# Autodesk Inventor assembly: Assembly
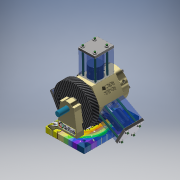
[picture p0: Inventor's stored thumbnail of the model, 180x180]
Saved by Autodesk Inventor 2017 (Build 210142000, 142)
## iProperties
Created: 2020-01-14
Part Number: Assembly
Document SubType Name: Assembly
Designer: Admin
Author: Admin
## Documents named in this file (26)
- D:\tech design 11\Radial Engine\Submission\Parts and Assembly\Assembly23.iam
- D:\tech design 11\Radial Engine\Submission\Parts and Assembly\crankcase.ipt
- D:\tech design 11\Radial Engine\Submission\Parts and Assembly\valve.ipt
- D:\tech design 11\Radial Engine\Submission\Parts and Assembly\valvecrank.ipt
- D:\tech design 11\Radial Engine\Submission\Parts and Assembly\valvehousing.ipt
- D:\tech design 11\Radial Engine\Submission\Parts and Assembly\locatingpin.ipt
- D:\tech design 11\Radial Engine\Submission\Parts and Assembly\cylinder...ipt
- D:\tech design 11\Radial Engine\Submission\Parts and Assembly\base.ipt
- D:\tech design 11\Radial Engine\Submission\Parts and Assembly\bearing.ipt
- D:\tech design 11\Radial Engine\Submission\Parts and Assembly\crankshaft.ipt
- D:\tech design 11\Radial Engine\Submission\Parts and Assembly\flywheel.ipt
- D:\tech design 11\Radial Engine\Assembly\hubpin.ipt
- D:\tech design 11\Radial Engine\Submission\Parts and Assembly\Piston.ipt
- D:\tech design 11\Radial Engine\Submission\Parts and Assembly\Crankcase Cover.ipt
- D:\tech design 11\Radial Engine\Submission\Parts and Assembly\Connecting Rod Hub.ipt
- D:\tech design 11\Radial Engine\Submission\Parts and Assembly\Connecting Rod.ipt
- D:\tech design 11\Radial Engine\Submission\Parts and Assembly\Wrist Pin.ipt
- D:\tech design 11\Radial Engine\Submission\Parts and Assembly\cylinderhead.ipt
- D:\tech design 11\Radial Engine\Submission\Parts and Assembly\enginefoot.ipt
- D:\tech design 11\Radial Engine\Submission\Parts and Assembly\studs.ipt
- D:\tech design 11\Radial Engine\parts\turningfixture.ipt
- D:\tech design 11\Radial Engine\Submission\Parts and Assembly\ventplug.ipt
- C:\Users\Admin\Documents\Inventor\Content Center Files\R2017\en-US\GB_T 70.1-2000\Screw GB_T 70.1 M3 x 14.ipt
- C:\Users\Admin\Documents\Inventor\Content Center Files\R2017\en-US\GB_T 70.1-2000\Screw GB_T 70.1 M3 x 5.ipt
- C:\Users\Admin\Documents\Inventor\Content Center Files\R2017\en-US\PN-87 M-82302\PN-87_M-82302 - M2 x 12.ipt
- C:\Users\Admin\Documents\Inventor\Content Center Files\R2017\en-US\CNS 3129\CNS 3129 - M 2 x 0.4.ipt
## Components (72 placed, 25 different names)
1. crankcase:1 — Insert:2, Insert:3, Insert:4, Insert:5, Insert:6, Insert:7, Mate:4, Insert:27, Mate:17, Insert:33, Insert:34, Mate:18, Mate:19, Insert:50, Mate:44
2. cylinder..:1 — Insert:2, Insert:3, Mate:11, Insert:19, Mate:14
3. cylinder..:2 — Insert:4, Insert:5, Mate:7, Insert:21, Mate:16
4. cylinder..:3 — Insert:6, Insert:7, Mate:5, Insert:20, Mate:15
5. base:1 — Mate:1, Insert:11, Insert:12, Mate:20, Mate:21, Mate:22, Mate:23, Mate:24, Mate:25, Mate:26, Mate:27
6. bearing:1 — Mate:1, Insert:11, Insert:12, Mate:2
7. crankshaft:1 — Mate:2, Mate:4, Rotation:1, Mate:42, Insert:72, Insert:73
8. Crankcase Cover:1 — Mate:19, Insert:51, Insert:52, Insert:53, Insert:54, Insert:55, Insert:56, Mate:44, Insert:72, Insert:74
9. Connecting Rod Hub:1 — Insert:68, Insert:69, Mate:42, Mate:43, Insert:70, Insert:71, Insert:73, Insert:75, Insert:76
10. Connecting Rod:1 — Cylindrical:3, Insert:69
11. Connecting Rod:2 — Cylindrical:1, Insert:68
12. Connecting Rod:3 — Cylindrical:2, Insert:70
13. Piston:1 — Mate:5, Mate:6, Mate:10
14. Piston:2 — Mate:7, Mate:8, Mate:9
15. Piston:3 — Mate:11, Mate:12, Mate:13
16. Wrist Pin:1 — Cylindrical:2, Mate:8, Mate:9
17. Wrist Pin:2 — Cylindrical:1, Mate:6, Mate:10
18. Wrist Pin:3 — Cylindrical:3, Mate:12, Mate:13
19. cylinderhead:1 — Insert:19, Mate:14, Insert:35, Insert:36, Insert:37, Insert:38, Insert:64, Insert:65, Insert:66, Insert:67
20. cylinderhead:2 — Insert:20, Mate:15, Insert:39, Insert:40, Insert:41, Insert:42, Mate:41, Insert:57, Insert:58, Insert:59
21. cylinderhead:3 — Insert:21, Mate:16, Insert:43, Insert:44, Insert:45, Insert:46, Insert:60, Insert:61, Insert:62, Insert:63
22. flywheel:1 — Rotation:1, Insert:74
23. valvecrank:1 — Insert:31, Mate:18, Insert:71
24. hubpin:1 — Mate:43
25. hubpin:2
26. hubpin:3 — Insert:75
27. enginefoot:1 — Insert:50
28. locatingpin:1 — Insert:47
29. studs:1 — Insert:37
30. valve:2 — Insert:31
31. valvehousing:1 — Mate:17, Insert:33, Insert:34, Insert:47, Mate:28, Mate:29, Mate:30, Mate:31, Mate:32, Mate:33, Mate:34, Mate:35, Mate:36, Mate:37, Mate:38, Mate:39
32. ventplug:1 — Insert:27
33. studs:2 — Insert:36
34. studs:3 — Insert:35
35. studs:4 — Insert:39, Mate:40
36. studs:5 — Insert:41
37. studs:6 — Insert:42
38. studs:10 — Insert:38
39. studs:11 — Insert:40
40. studs:12 — Insert:43
41. studs:13 — Insert:45
42. studs:17 — Insert:46
43. studs:19 — Insert:44
44. turningfixture:1
45. Screw GB/T 70.1-2000 M3 x 14:1 — Mate:20, Mate:21
46. Screw GB/T 70.1-2000 M3 x 14:2 — Mate:22, Mate:23
47. Screw GB/T 70.1-2000 M3 x 14:3 — Mate:24, Mate:25
48. Screw GB/T 70.1-2000 M3 x 5:1 — Mate:26, Mate:27
49. PN-87/M-82302 M2 x 12:1 — Mate:28, Mate:29
50. PN-87/M-82302 M2 x 12:2 — Mate:30, Mate:31
51. PN-87/M-82302 M2 x 12:3 — Mate:32, Mate:33
52. PN-87/M-82302 M2 x 12:4 — Mate:34, Mate:35
53. PN-87/M-82302 M2 x 12:5 — Mate:36, Mate:37
54. PN-87/M-82302 M2 x 12:6 — Mate:38, Mate:39
55. PN-87/M-82302 M2 x 12:7 — Insert:51
56. PN-87/M-82302 M2 x 12:8 — Insert:54
57. PN-87/M-82302 M2 x 12:9 — Insert:52
58. PN-87/M-82302 M2 x 12:11 — Insert:56
59. PN-87/M-82302 M2 x 12:12 — Insert:55, Insert:76
60. PN-87/M-82302 M2 x 12:13 — Insert:53
61. CNS 3129 M 2:1 — Mate:40, Mate:41
62. CNS 3129 M 2:2 — Insert:57
63. CNS 3129 M 2:3 — Insert:58
64. CNS 3129 M 2:4 — Insert:59
65. CNS 3129 M 2:5 — Insert:60
66. CNS 3129 M 2:6 — Insert:61
67. CNS 3129 M 2:7 — Insert:62
68. CNS 3129 M 2:8 — Insert:63
69. CNS 3129 M 2:9 — Insert:64
70. CNS 3129 M 2:10 — Insert:65
71. CNS 3129 M 2:11 — Insert:66
72. CNS 3129 M 2:12 — Insert:67
## Relationships (102: Insert 55, Mate 43, CylindricalJoint 3, RelateRotation 1)
- Insert:2: crankcase:1 ↔ cylinder..:1
- Insert:3: crankcase:1 ↔ cylinder..:1
- Insert:4: crankcase:1 ↔ cylinder..:2
- Insert:5: crankcase:1 ↔ cylinder..:2
- Insert:6: crankcase:1 ↔ cylinder..:3
- Insert:7: crankcase:1 ↔ cylinder..:3
- Mate:1: base:1 ↔ bearing:1
- Insert:11: base:1 ↔ bearing:1
- Insert:12: base:1 ↔ bearing:1
- Mate:2: bearing:1 ↔ crankshaft:1
- Mate:4: crankcase:1 ↔ crankshaft:1
- Mate:5: cylinder..:3 ↔ Piston:1
- Cylindrical:1: Connecting Rod:2 ↔ Wrist Pin:2
- Mate:6: Piston:1 ↔ Wrist Pin:2
- Mate:7: cylinder..:2 ↔ Piston:2
- Cylindrical:2: Connecting Rod:3 ↔ Wrist Pin:1
- Mate:8: Piston:2 ↔ Wrist Pin:1
- Mate:9: Piston:2 ↔ Wrist Pin:1
- Mate:10: Piston:1 ↔ Wrist Pin:2
- Cylindrical:3: Connecting Rod:1 ↔ Wrist Pin:3
- Mate:11: cylinder..:1 ↔ Piston:3
- Mate:12: Piston:3 ↔ Wrist Pin:3
- Mate:13: Piston:3 ↔ Wrist Pin:3
- Insert:19: cylinder..:1 ↔ cylinderhead:1
- Mate:14: cylinder..:1 ↔ cylinderhead:1
- Insert:20: cylinder..:3 ↔ cylinderhead:2
- Mate:15: cylinder..:3 ↔ cylinderhead:2
- Insert:21: cylinder..:2 ↔ cylinderhead:3
- Mate:16: cylinder..:2 ↔ cylinderhead:3
- Insert:27: crankcase:1 ↔ ventplug:1
- Insert:31: valvecrank:1 ↔ valve:2
- Rotation:1 [RelateRotation] (1 ul): crankshaft:1 ↔ flywheel:1
- Mate:17: crankcase:1 ↔ valvehousing:1
- Insert:33: crankcase:1 ↔ valvehousing:1
- Insert:34: crankcase:1 ↔ valvehousing:1
- Mate:18: crankcase:1 ↔ valvecrank:1
- Insert:35 (-2.54 mm): cylinderhead:1 ↔ studs:3
- Insert:36 (-2.54 mm): cylinderhead:1 ↔ studs:2
- Insert:37 (-2.54 mm): cylinderhead:1 ↔ studs:1
- Insert:38 (-2.54 mm): cylinderhead:1 ↔ studs:10
- Insert:39 (-2.54 mm): cylinderhead:2 ↔ studs:4
- Insert:40 (-2.54 mm): cylinderhead:2 ↔ studs:11
- Insert:41 (-2.54 mm): cylinderhead:2 ↔ studs:5
- Insert:42 (-2.54 mm): cylinderhead:2 ↔ studs:6
- Insert:43 (-2.54 mm): cylinderhead:3 ↔ studs:12
- Insert:44 (-2.54 mm): cylinderhead:3 ↔ studs:19
- Insert:45 (-2.54 mm): cylinderhead:3 ↔ studs:13
- Insert:46 (-2.54 mm): cylinderhead:3 ↔ studs:17
- Insert:47: locatingpin:1 ↔ valvehousing:1
- Mate:19: crankcase:1 ↔ Crankcase Cover:1
- Mate:20: base:1 ↔ Screw GB/T 70.1-2000 M3 x 14:1
- Mate:21: base:1 ↔ Screw GB/T 70.1-2000 M3 x 14:1
- Mate:22: base:1 ↔ Screw GB/T 70.1-2000 M3 x 14:2
- Mate:23: base:1 ↔ Screw GB/T 70.1-2000 M3 x 14:2
- Mate:24: base:1 ↔ Screw GB/T 70.1-2000 M3 x 14:3
- Mate:25: base:1 ↔ Screw GB/T 70.1-2000 M3 x 14:3
- Mate:26: base:1 ↔ Screw GB/T 70.1-2000 M3 x 5:1
- Mate:27: base:1 ↔ Screw GB/T 70.1-2000 M3 x 5:1
- Insert:50: crankcase:1 ↔ enginefoot:1
- Mate:28: valvehousing:1 ↔ PN-87/M-82302 M2 x 12:1
- Mate:29: valvehousing:1 ↔ PN-87/M-82302 M2 x 12:1
- Mate:30: valvehousing:1 ↔ PN-87/M-82302 M2 x 12:2
- Mate:31: valvehousing:1 ↔ PN-87/M-82302 M2 x 12:2
- Mate:32: valvehousing:1 ↔ PN-87/M-82302 M2 x 12:3
- Mate:33: valvehousing:1 ↔ PN-87/M-82302 M2 x 12:3
- Mate:34: valvehousing:1 ↔ PN-87/M-82302 M2 x 12:4
- Mate:35: valvehousing:1 ↔ PN-87/M-82302 M2 x 12:4
- Mate:36: valvehousing:1 ↔ PN-87/M-82302 M2 x 12:5
- Mate:37: valvehousing:1 ↔ PN-87/M-82302 M2 x 12:5
- Mate:38: valvehousing:1 ↔ PN-87/M-82302 M2 x 12:6
- Mate:39: valvehousing:1 ↔ PN-87/M-82302 M2 x 12:6
- Insert:51: Crankcase Cover:1 ↔ PN-87/M-82302 M2 x 12:7
- Insert:52: Crankcase Cover:1 ↔ PN-87/M-82302 M2 x 12:9
- Insert:53: Crankcase Cover:1 ↔ PN-87/M-82302 M2 x 12:13
- Insert:54: Crankcase Cover:1 ↔ PN-87/M-82302 M2 x 12:8
- Insert:55: Crankcase Cover:1 ↔ PN-87/M-82302 M2 x 12:12
- Insert:56: Crankcase Cover:1 ↔ PN-87/M-82302 M2 x 12:11
- Mate:40: studs:4 ↔ CNS 3129 M 2:1
- Mate:41: cylinderhead:2 ↔ CNS 3129 M 2:1
- Insert:57: cylinderhead:2 ↔ CNS 3129 M 2:2
- Insert:58: cylinderhead:2 ↔ CNS 3129 M 2:3
- Insert:59: cylinderhead:2 ↔ CNS 3129 M 2:4
- Insert:60: cylinderhead:3 ↔ CNS 3129 M 2:5
- Insert:61: cylinderhead:3 ↔ CNS 3129 M 2:6
- Insert:62: cylinderhead:3 ↔ CNS 3129 M 2:7
- Insert:63: cylinderhead:3 ↔ CNS 3129 M 2:8
- Insert:64: cylinderhead:1 ↔ CNS 3129 M 2:9
- Insert:65: cylinderhead:1 ↔ CNS 3129 M 2:10
- Insert:66: cylinderhead:1 ↔ CNS 3129 M 2:11
- Insert:67: cylinderhead:1 ↔ CNS 3129 M 2:12
- Insert:68: Connecting Rod Hub:1 ↔ Connecting Rod:2
- Insert:69: Connecting Rod Hub:1 ↔ Connecting Rod:1
- Mate:42: crankshaft:1 ↔ Connecting Rod Hub:1
- Mate:43: Connecting Rod Hub:1 ↔ hubpin:1
- Insert:70: Connecting Rod Hub:1 ↔ Connecting Rod:3
- Insert:71: Connecting Rod Hub:1 ↔ valvecrank:1
- Mate:44: crankcase:1 ↔ Crankcase Cover:1
- Insert:72: crankshaft:1 ↔ Crankcase Cover:1
- Insert:73: crankshaft:1 ↔ Connecting Rod Hub:1
- Insert:74: Crankcase Cover:1 ↔ flywheel:1
- Insert:75: Connecting Rod Hub:1 ↔ hubpin:3
- Insert:76: Connecting Rod Hub:1 ↔ PN-87/M-82302 M2 x 12:12
